# Autodesk Inventor assembly: COM-09939 - Rotary Potentiometer
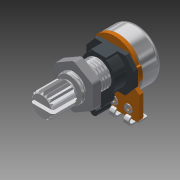
[picture p0: Inventor's stored thumbnail of the model, 180x180]
Saved by Autodesk Inventor 2014 SP1 (Build 180222100, 222)
## iProperties
Created: 2013-12-29
Part Number: COM-09939 - Rotary Potentiometer
Document SubType Name: Assembly
Designer: tom
Title: D:\My Documents\Work\GitHub\Component_Models\COM-09939 Rotary Pot\COM-09939 - Rotary Potentiometer.stp
Creation Date: 2013-12-29
Sending System: ACIS
Author: tom
## Documents named in this file (9)
- C:\Users\tom\Documents\GitHub\Component_Models\COM-09939 Rotary Pot\Inventor\COM-09939 - Rotary Potentiometer.iam
- C:\Users\tom\Documents\GitHub\Component_Models\COM-09939 Rotary Pot\Inventor\Component3.ipt
- C:\Users\tom\Documents\GitHub\Component_Models\COM-09939 Rotary Pot\Inventor\Component5.ipt
- C:\Users\tom\Documents\GitHub\Component_Models\COM-09939 Rotary Pot\Inventor\Component7.ipt
- C:\Users\tom\Documents\GitHub\Component_Models\COM-09939 Rotary Pot\Inventor\Component8.ipt
- C:\Users\tom\Documents\GitHub\Component_Models\COM-09939 Rotary Pot\Inventor\Component9.ipt
- C:\Users\tom\Documents\GitHub\Component_Models\COM-09939 Rotary Pot\Inventor\Component10.ipt
- C:\Users\tom\Documents\GitHub\Component_Models\COM-09939 Rotary Pot\Inventor\Component11.ipt
- C:\Users\tom\Documents\GitHub\Component_Models\COM-09939 Rotary Pot\Inventor\Nut.ipt
## Components (8 placed, 8 different names)
1. Component3
2. Component5
3. Component7
4. Component8 — Mate:1
5. Component9
6. Component10
7. Component11
8. Nut:1 — Mate:1
## Relationships (1: Mate 1)
- Mate:1: Component8 ↔ Nut:1
